# Autodesk Inventor assembly: Drive V3
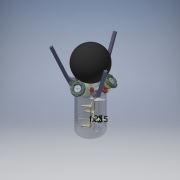
[picture p0: Inventor's stored thumbnail of the model, 180x180]
Saved by Autodesk Inventor 2019.1 (Build 231200000, 200)
## iProperties
Created: 2018-06-30
Part Number: Drive V3
Material: Generisch
Document SubType Name: Assembly
Designer: JochenAlt
Author: JochenAlt
## Documents named in this file (4)
- D:\Projects\Ondine\CAD\Drive V3.iam
- D:\Projects\Ondine\CAD\Sphere.ipt
- D:\Projects\Ondine\CAD\DriveChain V3.iam
- D:\Projects\Ondine\CAD\PCB\ControllerPCBHolder.ipt
## Components (5 placed, 3 different names)
1. Sphere:1 — Passend:38, Tangential:1
2. DriveChain V3:1 [sub-assembly] — Passend:41, Passend:47, Passend:48
3. DriveChain V3:2 [sub-assembly] — Passend:39, Tangential:1, Passend:46, Passend:49
4. DriveChain V3:3 [sub-assembly] — Passend:40, Passend:46, Passend:47
5. PCBHolder:1 — Passend:48, Passend:49
## Relationships (9: Mate 8, Tangent 1)
- Passend:38 [Mate]: Sphere:1
- Passend:39 [Mate]: DriveChain V3:2
- Passend:40 [Mate]: DriveChain V3:3
- Passend:41 [Mate]: DriveChain V3:1
- Tangential:1: Sphere:1 ↔ DriveChain V3:2
- Passend:46 [Mate]: DriveChain V3:2 ↔ DriveChain V3:3
- Passend:47 [Mate]: DriveChain V3:1 ↔ DriveChain V3:3
- Passend:48 [Mate]: DriveChain V3:1 ↔ PCBHolder:1
- Passend:49 [Mate]: DriveChain V3:2 ↔ PCBHolder:1
